# Autodesk Inventor assembly: Armature
(part 2 of 2)
- Affleurement:144 [Flush]: 1420-01-13 Noix M5:32 ↔ 1420-01-13 Noix M5:29
- Affleurement:145 [Flush]: 1420-01-13 Noix M5:31 ↔ 1420-01-13 Noix M5:29
- Affleurement:146 [Flush]: 1420-01-13 Noix M5:31 ↔ 1420-01-13 Noix M5:30
- Placage:186 [Mate]: 1420-01-13 Noix M5:32 ↔ Vis à tête percée - Métrique M5x0,8 x 12:19
- Placage:187 [Mate]: 1420-01-13 Noix M5:29 ↔ Vis à tête percée - Métrique M5x0,8 x 12:18
- Placage:188 [Mate]: 1420-01-13 Noix M5:31 ↔ Vis à tête percée - Métrique M5x0,8 x 12:20
- Placage:189 [Mate]: 1420-01-13 Noix M5:30 ↔ Vis à tête percée - Métrique M5x0,8 x 12:17
- Affleurement:147 [Flush]: 1420-01-13 Noix M5:31 ↔ 1420-01-13 Noix M5:30
- Affleurement:148 [Flush]: 1420-01-13 Noix M5:32 ↔ 1420-01-13 Noix M5:29
- Affleurement:149 [Flush]: 1420-01-13 Noix M5:32 ↔ 1420-01-13 Noix M5:30
- Affleurement:150 [Flush]: 1420-01-13 Noix M5:27 ↔ 1420-01-13 Noix M5:26
- Affleurement:151 [Flush]: 1420-01-13 Noix M5:28 ↔ 1420-01-13 Noix M5:25
- Affleurement:152 [Flush]: 1420-01-13 Noix M5:28 ↔ 1420-01-13 Noix M5:27
- Affleurement:153 [Flush]: 1420-01-13 Noix M5:30 ↔ 1420-01-13 Noix M5:27
- Placage:190 [Mate]: 1420-01-03 Profile horizontal 20x20x360:1 ↔ 1420-01-13 Noix M5:28
- Affleurement:154 [Flush]: 1420-01-13 Noix M5:40 ↔ 1420-01-13 Noix M5:37
- Affleurement:155 [Flush]: 1420-01-13 Noix M5:38 ↔ 1420-01-13 Noix M5:37
- Affleurement:156 [Flush]: 1420-01-13 Noix M5:40 ↔ 1420-01-13 Noix M5:39
- Placage:191 [Mate]: 1420-01-13 Noix M5:39 ↔ Vis à tête percée - Métrique M5x0,8 x 12:5
- Placage:192 [Mate]: 1420-01-13 Noix M5:37 ↔ Vis à tête percée - Métrique M5x0,8 x 12:6
- Placage:193 [Mate]: 1420-01-13 Noix M5:40 ↔ Vis à tête percée - Métrique M5x0,8 x 12:7
- Affleurement:157 [Flush]: 1420-01-13 Noix M5:36 ↔ 1420-01-13 Noix M5:33
- Affleurement:158 [Flush]: 1420-01-13 Noix M5:35 ↔ 1420-01-13 Noix M5:33
- Affleurement:159 [Flush]: 1420-01-13 Noix M5:34 ↔ 1420-01-13 Noix M5:33
- Placage:194 [Mate]: 1420-01-13 Noix M5:36 ↔ Vis à tête percée - Métrique M5x0,8 x 12:4
- Placage:195 [Mate]: 1420-01-13 Noix M5:35 ↔ Vis à tête percée - Métrique M5x0,8 x 12:1
- Placage:196 [Mate]: 1420-01-13 Noix M5:34 ↔ Vis à tête percée - Métrique M5x0,8 x 12:2
- Placage:197 [Mate]: 1420-01-13 Noix M5:33 ↔ Vis à tête percée - Métrique M5x0,8 x 12:3
- Placage:198 [Mate]: 1420-01-13 Noix M5:38 ↔ Vis à tête percée - Métrique M5x0,8 x 12:8
- Affleurement:160 [Flush]: 1420-01-13 Noix M5:38 ↔ 1420-01-13 Noix M5:37
- Affleurement:161 [Flush]: 1420-01-13 Noix M5:40 ↔ 1420-01-13 Noix M5:38
- Affleurement:162 [Flush]: 1420-01-13 Noix M5:39 ↔ 1420-01-13 Noix M5:37
- Placage:199 [Mate]: 1420-01-03 Profile horizontal 20x20x360:5 ↔ 1420-01-13 Noix M5:33
- Affleurement:163 [Flush]: 1420-01-13 Noix M5:35 ↔ 1420-01-13 Noix M5:33
- Affleurement:164 [Flush]: 1420-01-13 Noix M5:36 ↔ 1420-01-13 Noix M5:35
- Affleurement:165 [Flush]: 1420-01-13 Noix M5:34 ↔ 1420-01-13 Noix M5:33
- Affleurement:166 [Flush]: 1420-01-13 Noix M5:40 ↔ 1420-01-13 Noix M5:33
- Affleurement:167 [Flush]: 1420-01-13 Noix M5:43 ↔ 1420-01-13 Noix M5:41
- Affleurement:168 [Flush]: 1420-01-13 Noix M5:42 ↔ 1420-01-13 Noix M5:41
- Affleurement:169 [Flush]: 1420-01-13 Noix M5:44 ↔ 1420-01-13 Noix M5:42
- Affleurement:170 [Flush]: 1420-01-13 Noix M5:48 ↔ 1420-01-13 Noix M5:45
- Affleurement:171 [Flush]: 1420-01-13 Noix M5:47 ↔ 1420-01-13 Noix M5:46
- Affleurement:172 [Flush]: 1420-01-13 Noix M5:48 ↔ 1420-01-13 Noix M5:47
- Placage:200 [Mate]: 1420-01-13 Noix M5:48 ↔ Vis à tête percée - Métrique M5x0,8 x 12:15
- Placage:201 [Mate]: 1420-01-13 Noix M5:45 ↔ Vis à tête percée - Métrique M5x0,8 x 12:13
- Placage:202 [Mate]: 1420-01-13 Noix M5:42 ↔ Vis à tête percée - Métrique M5x0,8 x 12:12
- Placage:203 [Mate]: 1420-01-13 Noix M5:44 ↔ Vis à tête percée - Métrique M5x0,8 x 12:9
- Placage:204 [Mate]: 1420-01-13 Noix M5:43 ↔ Vis à tête percée - Métrique M5x0,8 x 12:10
- Placage:205 [Mate]: 1420-01-13 Noix M5:41 ↔ Vis à tête percée - Métrique M5x0,8 x 12:11
- Placage:206 [Mate]: 1420-01-13 Noix M5:46 ↔ Vis à tête percée - Métrique M5x0,8 x 12:14
- Placage:207 [Mate]: 1420-01-13 Noix M5:47 ↔ Vis à tête percée - Métrique M5x0,8 x 12:16
- Affleurement:173 [Flush]: 1420-01-13 Noix M5:45 ↔ 1420-01-13 Noix M5:43
- Placage:208 [Mate]: 1420-01-03 Profile horizontal 20x20x360:3 ↔ 1420-01-13 Noix M5:45
- Affleurement:174 [Flush]: 1420-01-13 Noix M5:46 ↔ 1420-01-13 Noix M5:45
- Affleurement:175 [Flush]: 1420-01-13 Noix M5:48 ↔ 1420-01-13 Noix M5:47
- Affleurement:176 [Flush]: 1420-01-13 Noix M5:47 ↔ 1420-01-13 Noix M5:46
- Affleurement:177 [Flush]: 1420-01-13 Noix M5:42 ↔ 1420-01-13 Noix M5:41
- Affleurement:178 [Flush]: 1420-01-13 Noix M5:44 ↔ 1420-01-13 Noix M5:42
- Affleurement:179 [Flush]: 1420-01-13 Noix M5:44 ↔ 1420-01-13 Noix M5:43
- Affleurement:180 [Flush]: DIN 7991 M4x10:1 ↔ DIN 7991 M4x10:2
- Placage:209 [Mate]: 1420-01-14 Coins inferieur:2 ↔ DIN 7991 M4x10:1
- Placage:210 [Mate]: 1420-01-14 Coins inferieur:2 ↔ DIN 7991 M4x10:2
- Affleurement:181 [Flush]: DIN 7991 M4x10:11 ↔ DIN 7991 M4x10:12
- Placage:212 [Mate]: 1420-01-15 Coins superieur:2 ↔ DIN 7991 M4x10:11
- Placage:213 [Mate]: 1420-01-15 Coins superieur:2 ↔ DIN 7991 M4x10:12
- Affleurement:182 [Flush]: DIN 7991 M4x10:3 ↔ DIN 7991 M4x10:4
- Placage:214 [Mate]: 1420-01-14 Coins inferieur:1 ↔ DIN 7991 M4x10:3
- Placage:215 [Mate]: 1420-01-14 Coins inferieur:1 ↔ DIN 7991 M4x10:4
- Affleurement:183 [Flush]: DIN 7991 M4x10:5 ↔ DIN 7991 M4x10:6
- Placage:216 [Mate]: 1420-01-14 Coins inferieur:3 ↔ DIN 7991 M4x10:5
- Placage:217 [Mate]: 1420-01-14 Coins inferieur:3 ↔ DIN 7991 M4x10:6
- Affleurement:184 [Flush]: DIN 7991 M4x10:7 ↔ DIN 7991 M4x10:8
- Placage:218 [Mate]: 1420-01-15 Coins superieur:3 ↔ DIN 7991 M4x10:8
- Placage:219 [Mate]: 1420-01-15 Coins superieur:3 ↔ DIN 7991 M4x10:7
- Affleurement:185 [Flush]: DIN 7991 M4x10:9 ↔ DIN 7991 M4x10:10
- Placage:220 [Mate]: 1420-01-15 Coins superieur:1 ↔ DIN 7991 M4x10:9
- Placage:221 [Mate]: 1420-01-15 Coins superieur:1 ↔ DIN 7991 M4x10:10
- Affleurement:186 [Flush]: 1420-01-12 Noix M4:9 ↔ 1420-01-12 Noix M4:10
- Placage:222 [Mate]: DIN 7991 M4x10:10 ↔ 1420-01-12 Noix M4:10
- Placage:223 [Mate]: DIN 7991 M4x10:9 ↔ 1420-01-12 Noix M4:9
- Affleurement:187 [Flush]: 1420-01-12 Noix M4:9 ↔ 1420-01-12 Noix M4:10
- Affleurement:188 [Flush]: 1420-01-12 Noix M4:6 ↔ 1420-01-12 Noix M4:5
- Placage:224 [Mate]: 1420-01-12 Noix M4:5 ↔ DIN 7991 M4x10:6
- Placage:225 [Mate]: 1420-01-12 Noix M4:6 ↔ DIN 7991 M4x10:5
- Affleurement:189 [Flush]: 1420-01-12 Noix M4:6 ↔ 1420-01-12 Noix M4:5
- Affleurement:190 [Flush]: 1420-01-12 Noix M4:4 ↔ 1420-01-12 Noix M4:3
- Placage:226 [Mate]: 1420-01-12 Noix M4:4 ↔ DIN 7991 M4x10:4
- Placage:227 [Mate]: 1420-01-12 Noix M4:3 ↔ DIN 7991 M4x10:3
- Affleurement:191 [Flush]: 1420-01-12 Noix M4:1 ↔ 1420-01-12 Noix M4:2
- Placage:228 [Mate]: DIN 7991 M4x10:8 ↔ 1420-01-12 Noix M4:1
- Placage:229 [Mate]: DIN 7991 M4x10:7 ↔ 1420-01-12 Noix M4:2
- Affleurement:192 [Flush]: 1420-01-12 Noix M4:11 ↔ 1420-01-12 Noix M4:12
- Placage:230 [Mate]: DIN 7991 M4x10:11 ↔ 1420-01-12 Noix M4:11
- Placage:231 [Mate]: DIN 7991 M4x10:12 ↔ 1420-01-12 Noix M4:12
- Affleurement:193 [Flush]: 1420-01-12 Noix M4:8 ↔ 1420-01-12 Noix M4:7
- Placage:232 [Mate]: 1420-01-12 Noix M4:7 ↔ DIN 7991 M4x10:2
- Placage:233 [Mate]: 1420-01-12 Noix M4:8 ↔ DIN 7991 M4x10:1
- Affleurement:194 [Flush]: 1420-01-12 Noix M4:8 ↔ 1420-01-12 Noix M4:7
- Affleurement:195 [Flush]: 1420-01-12 Noix M4:11 ↔ 1420-01-12 Noix M4:12
- Placage:234 [Mate]: 1420-01-01 Profile vertical 20x40x750:2 ↔ 1420-01-12 Noix M4:12
- Placage:235 [Mate]: 1420-01-15 Coins superieur:2 ↔ DIN 7991 M4x10:11
- Placage:236 [Mate]: 1420-01-14 Coins inferieur:2 ↔ DIN 7991 M4x10:1
- Placage:237 [Mate]: 1420-01-01 Profile vertical 20x40x750:2 ↔ 1420-01-12 Noix M4:8
- Placage:238 [Mate]: 1420-01-01 Profile vertical 20x40x750:3 ↔ 1420-01-12 Noix M4:5
- Placage:239 [Mate]: 1420-01-14 Coins inferieur:3 ↔ DIN 7991 M4x10:6
- Placage:240 [Mate]: 1420-01-01 Profile vertical 20x40x750:3 ↔ 1420-01-12 Noix M4:9
- Placage:241 [Mate]: 1420-01-15 Coins superieur:1 ↔ DIN 7991 M4x10:9
- Placage:242 [Mate]: 1420-01-01 Profile vertical 20x40x750:1 ↔ 1420-01-12 Noix M4:2
- Placage:243 [Mate]: 1420-01-15 Coins superieur:3 ↔ DIN 7991 M4x10:7
- Placage:244 [Mate]: 1420-01-01 Profile vertical 20x40x750:1 ↔ 1420-01-12 Noix M4:3
- Placage:245 [Mate]: 1420-01-14 Coins inferieur:1 ↔ DIN 7991 M4x10:4
- Affleurement:196 [Flush]: 1420-01-09 Pied:1 ↔ 1420-01-09 Pied:2
- Affleurement:197 [Flush]: 1420-01-09 Pied:2 ↔ 1420-01-09 Pied:3
- Placage:246 [Mate]: 1420-01-09 Pied:1 ↔ 1420-01-01 Profile vertical 20x40x750:2
- Placage:247 [Mate]: 1420-01-09 Pied:1 ↔ 1420-01-01 Profile vertical 20x40x750:2
- Placage:248 [Mate]: 1420-01-09 Pied:3 ↔ 1420-01-01 Profile vertical 20x40x750:3
- Placage:249 [Mate]: 1420-01-09 Pied:2 ↔ 1420-01-01 Profile vertical 20x40x750:1
- Affleurement:198 [Flush]: Vis à tête percée - Métrique M5x0,8 x 25:1 ↔ Vis à tête percée - Métrique M5x0,8 x 25:3
- Affleurement:199 [Flush]: Vis à tête percée - Métrique M5x0,8 x 25:1 ↔ Vis à tête percée - Métrique M5x0,8 x 25:2
- Placage:250 [Mate]: 1420-01-09 Pied:1 ↔ Vis à tête percée - Métrique M5x0,8 x 25:3
- Placage:251 [Mate]: 1420-01-09 Pied:1 ↔ Vis à tête percée - Métrique M5x0,8 x 25:3
- Placage:252 [Mate]: 1420-01-09 Pied:3 ↔ Vis à tête percée - Métrique M5x0,8 x 25:1
- Placage:253 [Mate]: 1420-01-09 Pied:2 ↔ Vis à tête percée - Métrique M5x0,8 x 25:2
